# Autodesk Inventor assembly: x-lift assembly
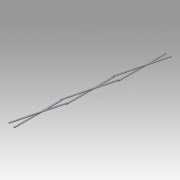
[picture p0: Inventor's stored thumbnail of the model, 180x180]
Saved by Autodesk Inventor 2016 (Build 200138000, 138)
## iProperties
Created: 2015-12-16
Part Number: x-lift assembly
Document SubType Name: Assembly
Designer: Delta
Author: Delta
## Documents named in this file (2)
- C:\Robotics\CAD\2015-16\custom cad parts\x-lift assembly.iam
- C:\Robotics\CAD\2015-16\custom cad parts\x-lift arm prototype piece.ipt
## Components (6 placed, 1 different names)
1. x-lift arm prototype piece:1 — Insert:1, Insert:3
2. x-lift arm prototype piece:2 — Insert:1, Insert:2
3. x-lift arm prototype piece:3 — Insert:2, Insert:4, Insert:5
4. x-lift arm prototype piece:4 — Insert:3, Insert:4, Insert:6
5. x-lift arm prototype piece:5 — Insert:5, Insert:7
6. x-lift arm prototype piece:6 — Insert:6, Insert:7
## Relationships (7: Insert 7)
- Insert:1: x-lift arm prototype piece:1 ↔ x-lift arm prototype piece:2
- Insert:2: x-lift arm prototype piece:2 ↔ x-lift arm prototype piece:3
- Insert:3: x-lift arm prototype piece:1 ↔ x-lift arm prototype piece:4
- Insert:4: x-lift arm prototype piece:3 ↔ x-lift arm prototype piece:4
- Insert:5: x-lift arm prototype piece:3 ↔ x-lift arm prototype piece:5
- Insert:6: x-lift arm prototype piece:4 ↔ x-lift arm prototype piece:6
- Insert:7: x-lift arm prototype piece:5 ↔ x-lift arm prototype piece:6
